# Autodesk Inventor assembly: Expand Spring 1
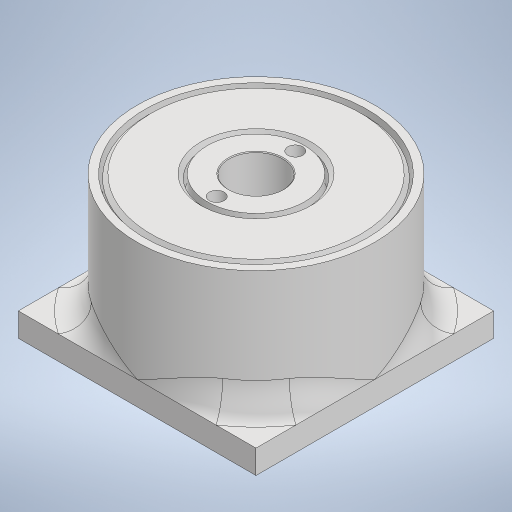
[picture p0: Inventor's stored thumbnail of the model, 512x512]
Saved by Autodesk Inventor 2023.4 (Build 274418000, 418)
## iProperties
Created: 2024-05-29
Part Number: Expand Spring 1
Document SubType Name: Assembly
Designer: Nathan Cai
Author: Nathan Cai
## Documents named in this file (4)
- E:\Documents\Inventor\Misc\Expand Spring\Expand Spring 1.iam
- E:\Documents\Inventor\Misc\Expand Spring\Base.ipt
- E:\Documents\Inventor\Misc\Expand Spring\Core.ipt
- E:\Documents\Inventor\Misc\Expand Spring\Cap.ipt
## Components (3 placed, 3 different names)
1. Base:1 — Mate:1, Mate:2, Mate:3, Flush:1
2. Core:1 — Mate:1, Mate:2
3. Cap:1 — Mate:3, Flush:1
## Relationships (4: Mate 3, Flush 1)
- Mate:1: Base:1 ↔ Core:1
- Mate:2: Base:1 ↔ Core:1
- Mate:3: Base:1 ↔ Cap:1
- Flush:1: Base:1 ↔ Cap:1
